# Autodesk Inventor assembly: sled
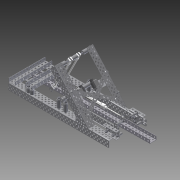
[picture p0: Inventor's stored thumbnail of the model, 180x180]
Saved by Autodesk Inventor 2014 SP1 (Build 180222100, 222)
## iProperties
Created: 2014-02-27
Part Number: sled
Document SubType Name: Assembly
Designer: Ryan
Author: Ryan
## Documents named in this file (36)
- C:\Users\Ryan\Desktop\sw\toss up 5th A bot\intake\sled.iam
- C:\Users\Ryan\Desktop\sw\lib\Aperture VEX CAD Library\Standoffs\BEAM-0500.ipt
- C:\Users\Ryan\Desktop\sw\lib\Aperture VEX CAD Library\Spacers\SPACER-0500-0125.ipt
- C:\Users\Ryan\Desktop\sw\lib\Aperture VEX CAD Library\Metal\C Channel\2 x 11.ipt
- C:\Users\Ryan\Desktop\sw\lib\Aperture VEX CAD Library\Metal\vex hinge\hinge.iam
- C:\Users\Ryan\Desktop\sw\lib\Aperture VEX CAD Library\Metal\C Channel\2 x 35.ipt
- C:\Users\Ryan\Desktop\sw\lib\Aperture VEX CAD Library\Spacers\SPACER-0500-0500.ipt
- C:\Users\Ryan\Desktop\sw\lib\Aperture VEX CAD Library\Metal\L Bar\2 x 14.ipt
- C:\Users\Ryan\Desktop\sw\lib\Aperture VEX CAD Library\Hardware\8-32\8-32_.375.ipt
- C:\Users\Ryan\Desktop\sw\lib\Aperture VEX CAD Library\Metal\Custom 1 bar\4 holes.ipt
- C:\Users\Ryan\Desktop\sw\lib\Aperture VEX CAD Library\Bearing Blocks\Bearing Block.ipt
- C:\Users\Ryan\Desktop\sw\lib\Aperture VEX CAD Library\Metal\Custom 1 bar\12.ipt
- C:\Users\Ryan\Desktop\sw\lib\Aperture VEX CAD Library\Pnuematics\Solenoid, Fwd, Reverse.iam
- C:\Users\Ryan\Desktop\sw\lib\Aperture VEX CAD Library\Shaft\5.5 inch shaft.ipt
- C:\Users\Ryan\Desktop\sw\lib\Aperture VEX CAD Library\Pnuematics\Cylinder, Bi-directional.iam
- C:\Users\Ryan\Desktop\sw\lib\Aperture VEX CAD Library\Pnuematics\End Gusset Fixed.ipt
- C:\Users\Ryan\Desktop\sw\lib\Aperture VEX CAD Library\Pnuematics\Cylinder, Bi-directional-Parts\Nut 8-32 Hex.ipt
- C:\Users\Ryan\Desktop\sw\lib\Aperture VEX CAD Library\Spacers\SPACER-0500-0250.ipt
- C:\Users\Ryan\Desktop\sw\lib\Aperture VEX CAD Library\Metal\Gussets\Lockbar.ipt
- C:\Users\Ryan\Desktop\sw\lib\Aperture VEX CAD Library\Spacers\SPACER-0500-0375.ipt
- C:\Users\Ryan\Desktop\sw\lib\Aperture VEX CAD Library\Hardware\8-32\8-32 nylock.ipt
- C:\Users\Ryan\Desktop\sw\lib\Aperture VEX CAD Library\Hardware\8-32\8-32_.500.ipt
- C:\Users\Ryan\Desktop\sw\lib\Aperture VEX CAD Library\Hardware\6-32\6-32_.250.ipt
- C:\Users\Ryan\Desktop\sw\lib\Aperture VEX CAD Library\Hardware\6-32\thinner locknut.iam
- C:\Users\Ryan\Desktop\sw\lib\Aperture VEX CAD Library\Spacers\thin\SPACER-0320-00625.ipt
- C:\Users\Ryan\Desktop\sw\lib\Aperture VEX CAD Library\Bearing Blocks\Pillow Block.ipt
- C:\Users\Ryan\Desktop\sw\lib\Aperture VEX CAD Library\Hardware\Shaft Collar.ipt
- C:\Users\Ryan\Desktop\sw\lib\Aperture VEX CAD Library\Metal\C Channel\2 x 4.ipt
- C:\Users\Ryan\Desktop\sw\lib\Aperture VEX CAD Library\Hardware\8-32\8-23_.750.ipt
- C:\Users\Ryan\Desktop\sw\lib\Aperture VEX CAD Library\Spacers\thin\SPACER-0320-0500.ipt
- C:\Users\Ryan\Desktop\sw\lib\Aperture VEX CAD Library\Spacers\thin\SPACER-0320-0250.ipt
- C:\Users\Ryan\Desktop\sw\lib\Aperture VEX CAD Library\Metal\C Channel\2 x 13 sides cut off.ipt
- C:\Users\Ryan\Desktop\sw\lib\Aperture VEX CAD Library\Metal\Custom 1 bar\1 x 3.ipt
- C:\Users\Ryan\Desktop\sw\lib\Aperture VEX CAD Library\Spacers\thin\SPACER-0320-0125.ipt
- C:\Users\Ryan\Desktop\sw\lib\Aperture VEX CAD Library\Spacers\thin\SPACER-0320-0375.ipt
- C:\Users\Ryan\Desktop\sw\lib\Aperture VEX CAD Library\Metal\L Bar\2 x 30.ipt
## Components (188 placed, 35 different names)
1. 2 x 30:1 — Mate:6, Flush:1, Flush:2, Mate:29, Mate:31, Mate:32, Mate:133, Mate:217, Mate:219, Mate:244, Mate:247, Mate:400, Mate:401, Mate:402, Mate:420, Mate:421, Mate:422, Mate:423, Mate:426, Mate:476, Flush:19, Flush:20, Mate:477, Mate:529, Mate:530, Mate:531, Mate:532
2. 2 x 11:1 — Mate:6, Flush:1, Flush:2, Mate:8, Mate:9, Flush:7, Flush:8, Mate:224, Flush:17, Flush:18
3. 2 x 30:2 — Mate:8, Mate:15, Mate:17, Mate:20, Mate:39, Mate:43, Mate:44, Mate:52, Mate:54, Mate:214, Mate:215, Mate:237, Mate:238, Mate:355, Mate:356, Mate:416, Mate:419, Flush:17, Flush:18, Flush:23, Mate:519, Flush:24, Mate:523, Mate:526, Mate:527, Mate:528, Mate:535
4. hinge:1 [sub-assembly] — Mate:9, Flush:7, Flush:8, Mate:10, Flush:9, Flush:10, Mate:94, Mate:95, Mate:96, Mate:136, Mate:137, Mate:192, Mate:220, Mate:221, Mate:222, Mate:404, Mate:408
5. 2 x 35:3 — Mate:10, Flush:9, Flush:10, Flush:12, Mate:277, Mate:279, Mate:306, Mate:307, Mate:309, Mate:312, Mate:322, Mate:323, Mate:324, Mate:327, Mate:403, Mate:409
6. SPACER-0500-0500:1 — Mate:15, Mate:17, Mate:23, Mate:24, Mate:212
7. SPACER-0500-0500:2 — Mate:20, Mate:21, Mate:22, Mate:213, Mate:258, Mate:416, Mate:417, Mate:418, Mate:419
8. SPACER-0500-0125:3 — Mate:21, Mate:22
9. SPACER-0500-0125:4 — Mate:23, Mate:24, Mate:35, Mate:36, Mate:37
10. SPACER-0500-0500:3 — Mate:29, Mate:31, Mate:216, Mate:422
11. SPACER-0500-0500:4 — Mate:32, Mate:218, Mate:420, Mate:421
12. SPACER-0500-0125:5 — Mate:261
13. SPACER-0500-0125:6 — Mate:260
14. 2 x 11:2 — Mate:35, Mate:36, Mate:37, Mate:257, Mate:259, Mate:262, Mate:263, Mate:417, Mate:418
15. 2 x 14:1 — Mate:39, Mate:40, Mate:41, Mate:42, Mate:45, Mate:56, Mate:57, Mate:58, Mate:59, Mate:60, Mate:64, Mate:65, Mate:66, Mate:67, Mate:68, Angle:1, Flush:11, Mate:151, Mate:241, Mate:242, Mate:254, Mate:289, Mate:291, Mate:299, Mate:475
16. 8-32_.375:1 — Mate:40, Mate:41, Mate:42, Mate:43, Mate:44, Mate:134, Mate:239
17. 4 holes:1 — Mate:45, Mate:46, Mate:47, Mate:49, Mate:51, Mate:53, Mate:55
18. 8-32_.375:2 — Mate:46, Mate:47, Mate:49, Mate:255, Mate:475
19. 8-32_.375:3 — Mate:51, Mate:52, Mate:53, Mate:54, Mate:55, Mate:135, Mate:236
20. Bearing Block:1 — Mate:56, Mate:57, Mate:58, Mate:59, Mate:69, Mate:70, Mate:75, Mate:92, Mate:284, Mate:285, Mate:286, Mate:287, Mate:288, Mate:290
21. 12:1 — Mate:60, Mate:61, Mate:62, Mate:63, Mate:144, Mate:145, Mate:146
22. 8-32_.375:4 — Mate:61, Mate:62, Mate:63, Mate:64, Mate:65, Mate:240
23. Solenoid, Fwd, Reverse:1 [sub-assembly] — Mate:66, Mate:67, Mate:68, Angle:1, Angle:5, Mate:298, Mate:300
24. 5.5 inch shaft:1 — Flush:11, Mate:69, Mate:70
25. Cylinder, Bi-directional:1 [sub-assembly] — Mate:75, Mate:76, Mate:77, Mate:78, Mate:87, Mate:93
26. Nut 8-32 Hex:1 — Mate:185, Mate:186
27. End Gusset Fixed:2 — Mate:76, Mate:77, Mate:78, Mate:86, Mate:325, Mate:326, Mate:327, Mate:330, Mate:332
28. Nut 8-32 Hex:2 — Mate:86, Mate:87
29. SPACER-0500-0500:5 — Mate:88, Mate:89, Mate:90
30. SPACER-0500-0500:6 — Mate:89, Mate:91, Mate:92, Mate:93, Mate:132
31. SPACER-0500-0250:1 — Mate:88, Mate:90, Mate:91
32. Lockbar:1 — Mate:94, Mate:95, Mate:96, Mate:200, Mate:201, Angle:6
33. 2 x 14:2 — Mate:97, Mate:98, Mate:99, Mate:100, Mate:101, Mate:103, Mate:109, Mate:110, Mate:111, Mate:112, Mate:113, Angle:3, Mate:115, Mate:116, Mate:133, Mate:138, Mate:142, Mate:143, Mate:150, Mate:248, Mate:251, Mate:253, Mate:294, Mate:295, Mate:297
34. 8-32_.375:5 — Mate:97, Mate:98, Mate:99, Mate:134, Mate:246
35. 4 holes:2 — Mate:100, Mate:102, Mate:104, Mate:105, Mate:106, Mate:107, Mate:108
36. 8-32_.375:6 — Mate:101, Mate:102, Mate:103, Mate:104, Mate:105, Mate:250
37. 8-32_.375:7 — Mate:106, Mate:107, Mate:108, Mate:135, Mate:245
38. Bearing Block:2 — Mate:109, Mate:110, Mate:111, Mate:112, Mate:117, Mate:124, Mate:280, Mate:281, Mate:282, Mate:283, Mate:292, Mate:293
39. 12:2 — Mate:113, Mate:139, Mate:140, Mate:141, Mate:147, Mate:148, Mate:149
40. Solenoid, Fwd, Reverse:2 [sub-assembly] — Angle:3, Mate:115, Mate:116, Mate:138, Angle:5, Mate:296, Mate:302
41. Cylinder, Bi-directional:2 [sub-assembly] — Mate:117, Mate:118, Mate:119, Mate:120, Mate:123, Mate:132, Mate:185, Mate:334
42. End Gusset Fixed:3 — Mate:118, Mate:119, Mate:120, Mate:186, Mate:304, Mate:305, Mate:315, Mate:318
43. SPACER-0500-0500:7 — Mate:125, Mate:127, Mate:128, Mate:333
44. SPACER-0500-0500:8 — Mate:123, Mate:124, Mate:125, Mate:126
45. SPACER-0500-0250:2 — Mate:126, Mate:127, Mate:128
46. Lockbar:2 — Mate:136, Mate:137, Mate:189, Mate:192, Mate:193, Mate:202, Mate:203, Angle:6
47. 8-32_.375:8 — Mate:139, Mate:140, Mate:141, Mate:142, Mate:143, Mate:249
48. 8-32_.375:9 — Mate:144, Mate:145, Mate:146, Mate:150, Mate:252
49. 8-32_.375:10 — Mate:147, Mate:148, Mate:149, Mate:151, Mate:243
50. SPACER-0500-0375:1 — Mate:333, Mate:334, Mate:335, Mate:336
51. 8-32_.375:22 — Mate:200, Mate:201, Mate:276
52. 8-32_.375:23 — Mate:202, Mate:203, Mate:278, Mate:403
53. 8-32_.375:26 — Mate:304, Mate:305, Mate:306, Mate:307, Mate:308, Mate:310, Mate:311, Mate:314
54. 8-32_.375:27 — Mate:268, Mate:320, Mate:321, Mate:322, Mate:323, Mate:325, Mate:326, Mate:331
55. 8-32_.375:28 — Mate:212, Mate:215, Mate:256
56. 8-32_.375:29 — Mate:213, Mate:214
57. 8-32_.375:30 — Mate:216, Mate:217
58. 8-32_.375:31 — Mate:218, Mate:219
59. 8-32 nylock:8 — Mate:236, Mate:237
60. 8-32 nylock:9 — Mate:238, Mate:239
61. 8-32 nylock:10 — Mate:240, Mate:241
62. 8-32 nylock:11 — Mate:242, Mate:243
63. 8-32 nylock:12 — Mate:244, Mate:245
64. 8-32 nylock:13 — Mate:246, Mate:247
65. 8-32 nylock:14 — Mate:248, Mate:249
66. 8-32 nylock:15 — Mate:250, Mate:251
67. 8-32 nylock:16 — Mate:252, Mate:253
68. 8-32 nylock:17 — Mate:254, Mate:255
69. 8-32 nylock:18 — Mate:256, Mate:257
70. 8-32 nylock:19 — Mate:258, Mate:259
71. 8-32 nylock:20 — Mate:260, Mate:263
72. 8-32 nylock:21 — Mate:261, Mate:262
73. 8-32 nylock:24 — Mate:268, Mate:332
74. 8-32 nylock:34 — Mate:276, Mate:277
75. 8-32 nylock:35 — Mate:278, Mate:279
76. 8-32 nylock:36 — Mate:280, Mate:281
77. 8-32 nylock:37 — Mate:282, Mate:283
78. 8-32 nylock:38 — Mate:284, Mate:285
79. 8-32 nylock:39 — Mate:286, Mate:287
80. 8-32_.500:1 — Mate:288, Mate:289
81. 8-32_.500:2 — Mate:290, Mate:291
82. 8-32_.500:3 — Mate:293, Mate:295
83. 8-32_.500:4 — Mate:292, Mate:294
84. 6-32_.250:1 — Mate:296, Mate:297, Mate:303
85. 6-32_.250:2 — Mate:298, Mate:299, Mate:301
86. thinner locknut:1 [sub-assembly] — Mate:300, Mate:301
87. thinner locknut:2 [sub-assembly] — Mate:302, Mate:303
88. SPACER-0320-00625:1 — Mate:308, Mate:309, Mate:310
89. SPACER-0320-00625:2 — Mate:311, Mate:312, Mate:316, Mate:317
90. 8-32 nylock:40 — Mate:314, Mate:315
91. SPACER-0320-00625:3 — Mate:316, Mate:317, Mate:318
92. SPACER-0320-00625:4 — Mate:320, Mate:321, Mate:324
93. SPACER-0320-00625:5 — Mate:331
94. SPACER-0320-00625:6 — Mate:330
95. SPACER-0500-0375:2 — Mate:335, Mate:336
96. Pillow Block:1 — Mate:358, Mate:359, Mate:360, Mate:361, Mate:362, Mate:363
97. SPACER-0500-0500:10
98. SPACER-0500-0500:12
99. SPACER-0500-0500:9
100. SPACER-0500-0500:11
101. 8-32_.375:46 — Mate:355
102. 8-32_.375:47 — Mate:356
103. 8-32 nylock:41 — Mate:358, Mate:359
104. 8-32 nylock:42 — Mate:360, Mate:361
105. SPACER-0500-0500:13 — Mate:362, Mate:363, Mate:365, Mate:366
106. SPACER-0500-0500:14 — Mate:364, Mate:365, Mate:367, Mate:368, Mate:369
107. SPACER-0500-0500:15 — Mate:364, Mate:366, Mate:367
108. Shaft Collar:1 — Mate:368, Mate:369, Mate:370, Mate:371
109. SPACER-0500-0125:7 — Mate:370, Mate:371, Mate:372, Mate:373
110. Cylinder, Bi-directional:3 [sub-assembly] — Mate:372, Mate:373, Mate:396, Mate:397, Mate:411, Mate:412, Mate:413, Mate:414
111. Pillow Block:2 — Mate:374, Mate:375, Mate:376, Mate:377, Mate:378, Mate:382, Mate:383, Mate:387, Mate:398, Mate:399
112. 8-32_.375:48 — Mate:379, Mate:401
113. 8-32_.375:49 — Mate:384, Mate:402
114. 8-32 nylock:43 — Mate:374, Mate:375
115. 8-32 nylock:44 — Mate:376, Mate:377
116. SPACER-0500-0500:16 — Mate:378, Mate:380, Mate:381, Mate:399
117. SPACER-0500-0500:17 — Mate:379, Mate:380, Mate:381, Mate:400
118. SPACER-0500-0500:18 — Mate:382, Mate:383, Mate:385, Mate:386
119. SPACER-0500-0500:19 — Mate:384, Mate:385, Mate:386
120. SPACER-0500-0500:20 — Mate:387, Mate:388, Mate:390, Mate:398
121. SPACER-0500-0500:21 — Mate:388, Mate:389, Mate:391, Mate:392, Mate:393, Mate:396
122. SPACER-0500-0500:22 — Mate:389, Mate:390, Mate:391
123. Shaft Collar:2 — Mate:392, Mate:393, Mate:394, Mate:395
124. SPACER-0500-0125:8 — Mate:394, Mate:395, Mate:397
125. 8-32 nylock:45 — Mate:404, Mate:405
126. 8-32 nylock:46 — Mate:407, Mate:408
127. 8-32 nylock:47 — Mate:406, Mate:409
128. End Gusset Fixed:4 — Mate:412, Mate:413, Mate:414, Mate:415, Mate:474, Mate:478
129. Nut 8-32 Hex:3 — Mate:411, Mate:415
130. 2 x 4:1 — Mate:423, Mate:424, Mate:428, Mate:430, Mate:435, Mate:436, Mate:437, Mate:439, Mate:440, Mate:441, Mate:444, Mate:476, Flush:19, Flush:20
131. 8-32 nylock:51 — Mate:437, Mate:438
132. SPACER-0320-0500:1 — Mate:430, Mate:433, Mate:434, Mate:435, Mate:436
133. 8-23_.750:1 — Mate:433, Mate:434, Mate:438
134. 8-32 nylock:52 — Mate:439, Mate:440, Mate:441, Mate:445
135. SPACER-0320-00625:7 — Mate:442, Mate:443, Mate:448
136. SPACER-0320-0250:1 — Mate:442, Mate:443, Mate:444, Mate:445
137. 8-23_.750:2 — Mate:449, Mate:450
138. 2 x 13 sides cut off:1 — Mate:448, Mate:449, Mate:450, Mate:451, Flush:15, Flush:16, Mate:453, Mate:455, Mate:457, Mate:463, Mate:465
139. 1 x 3:1 — Mate:451, Flush:15, Flush:16, Mate:452, Mate:454, Mate:456, Mate:459, Mate:461, Mate:466, Mate:468, Mate:469
140. SPACER-0320-0125:1 — Mate:452, Mate:453, Mate:454, Mate:460
141. SPACER-0320-0125:2 — Mate:455, Mate:456, Mate:457, Mate:458
142. 8-32_.375:52 — Mate:458, Mate:459, Mate:462
143. 8-32_.375:53 — Mate:460, Mate:461, Mate:464
144. 8-32 nylock:53 — Mate:462, Mate:463
145. 8-32 nylock:54 — Mate:464, Mate:465
146. SPACER-0320-0375:1 — Mate:466, Mate:468, Mate:469, Mate:470, Mate:471, Mate:472, Mate:525
147. 8-32 nylock:55 — Mate:470, Mate:473, Mate:474, Mate:478
148. BEAM-0500:3 — Mate:471, Mate:472, Mate:473
149. 2 x 4:2 — Mate:479, Mate:480, Mate:482, Mate:483, Mate:484, Mate:485, Mate:489, Mate:490, Mate:491, Mate:493, Flush:23, Mate:519, Flush:24
150. 8-32 nylock:57 — Mate:482, Mate:486
151. SPACER-0320-0500:2 — Mate:483, Mate:484, Mate:485, Mate:487, Mate:488
152. 8-23_.750:3 — Mate:486, Mate:487, Mate:488
153. 8-32 nylock:58 — Mate:489, Mate:490, Mate:491, Mate:492
154. SPACER-0320-0250:2 — Mate:492, Mate:493, Mate:494, Mate:520, Mate:521
155. 8-23_.750:4 — Mate:494, Mate:495, Mate:496, Mate:524
156. 2 x 13 sides cut off:2 — Mate:495, Mate:496, Flush:21, Flush:22, Mate:497, Mate:499, Mate:501, Mate:503, Mate:508, Mate:510, Mate:522, Mate:524
157. 1 x 3:2 — Flush:21, Flush:22, Mate:497, Mate:498, Mate:500, Mate:502, Mate:504, Mate:506, Mate:512, Mate:513, Mate:514
158. SPACER-0320-0125:3 — Mate:498, Mate:499, Mate:500, Mate:507
159. SPACER-0320-0125:4 — Mate:501, Mate:502, Mate:503, Mate:505
160. 8-32_.375:55 — Mate:504, Mate:505, Mate:509
161. 8-32_.375:56 — Mate:506, Mate:507, Mate:511
162. 8-32 nylock:59 — Mate:508, Mate:509
163. 8-32 nylock:60 — Mate:510, Mate:511
164. SPACER-0320-0375:2 — Mate:512, Mate:513, Mate:514, Mate:515, Mate:517, Mate:518, Mate:525
165. 8-32 nylock:61 — Mate:515, Mate:516
166. BEAM-0500:4 — Mate:516, Mate:517, Mate:518
167. SPACER-0320-00625:8 — Mate:520, Mate:521, Mate:522
168. 8-32 nylock:63 — Mate:526, Mate:527, Mate:528, Mate:534
169. 8-32 nylock:64 — Mate:529, Mate:530, Mate:531, Mate:533
170. SPACER-0320-00625:9 — Mate:532, Mate:533
171. SPACER-0320-00625:10 — Mate:534, Mate:535
172. 8-32_.375:32 — Mate:220, Mate:221, Mate:222, Mate:223
173. 8-32_.375:12 — Mate:189, Mate:193, Mate:407
174. 8-32 nylock:1 — Mate:223, Mate:224
175. 8-32_.375:40
176. 8-32_.375:41 — Mate:406
177. 8-32 nylock:6
178. 8-32_.375:42
179. 8-32_.375:43 — Mate:405
180. 8-32 nylock:7
181. 8-32_.375:50 — Mate:424, Mate:426, Mate:427, Mate:477
182. 8-32 nylock:48 — Mate:427, Mate:428
183. 8-32_.375:51
184. 8-32 nylock:49
185. 8-32_.375:54 — Mate:479, Mate:481, Mate:523
186. 8-32 nylock:56 — Mate:480, Mate:481
187. 8-32_.375:57
188. 8-32 nylock:62
## Component patterns: (3 elements, first: 8-32_.375:32 + 8-32_.375:12 + 8-32 nylock:1), (2 elements, first: 8-32_.375:50 + 8-32 nylock:48), (2 elements, first: 8-32_.375:54 + 8-32 nylock:56)
## Relationships (436: Mate 414, Flush 18, Angle 4)
- Mate:6: 2 x 30:1 ↔ 2 x 11:1
- Flush:1: 2 x 30:1 ↔ 2 x 11:1
- Flush:2: 2 x 30:1 ↔ 2 x 11:1
- Mate:8: 2 x 11:1 ↔ 2 x 30:2
- Mate:9: 2 x 11:1 ↔ hinge:1
- Flush:7: 2 x 11:1 ↔ hinge:1
- Flush:8: 2 x 11:1 ↔ hinge:1
- Mate:10: hinge:1 ↔ 2 x 35:3
- Flush:9: hinge:1 ↔ 2 x 35:3
- Flush:10: hinge:1 ↔ 2 x 35:3
- Mate:15: 2 x 30:2 ↔ SPACER-0500-0500:1
- Mate:17 (2.3114 mm): 2 x 30:2 ↔ SPACER-0500-0500:1
- Mate:20: 2 x 30:2 ↔ SPACER-0500-0500:2
- Mate:21: SPACER-0500-0500:2 ↔ SPACER-0500-0125:3
- Mate:22: SPACER-0500-0500:2 ↔ SPACER-0500-0125:3
- Mate:23: SPACER-0500-0500:1 ↔ SPACER-0500-0125:4
- Mate:24: SPACER-0500-0500:1 ↔ SPACER-0500-0125:4
- [Mate]: SPACER-0500-0500:4 ↔ SPACER-0500-0125:5
- [Mate]: SPACER-0500-0500:4 ↔ SPACER-0500-0125:5
- [Mate]: SPACER-0500-0500:3 ↔ SPACER-0500-0125:6
- [Mate]: SPACER-0500-0500:3 ↔ SPACER-0500-0125:6
- Mate:29 (2.3114 mm): 2 x 30:1 ↔ SPACER-0500-0500:3
- Mate:31: 2 x 30:1 ↔ SPACER-0500-0500:3
- Mate:32: 2 x 30:1 ↔ SPACER-0500-0500:4
- Mate:35: SPACER-0500-0125:4 ↔ 2 x 11:2
- Mate:36 (2.3114 mm): SPACER-0500-0125:4 ↔ 2 x 11:2
- Mate:37 (2.3114 mm): SPACER-0500-0125:4 ↔ 2 x 11:2
- Mate:39: 2 x 30:2 ↔ 2 x 14:1
- Mate:40 (2.3114 mm): 2 x 14:1 ↔ 8-32_.375:1
- Mate:41 (2.3114 mm): 2 x 14:1 ↔ 8-32_.375:1
- Mate:42: 2 x 14:1 ↔ 8-32_.375:1
- Mate:43 (2.3114 mm): 2 x 30:2 ↔ 8-32_.375:1
- Mate:44 (-61.1886 mm): 2 x 30:2 ↔ 8-32_.375:1
- Mate:45: 2 x 14:1 ↔ 4 holes:1
- Mate:46 (2.3114 mm): 4 holes:1 ↔ 8-32_.375:2
- Mate:47 (2.3114 mm): 4 holes:1 ↔ 8-32_.375:2
- Mate:49: 4 holes:1 ↔ 8-32_.375:2
- Mate:51 (2.3114 mm): 4 holes:1 ↔ 8-32_.375:3
- Mate:52 (65.8114 mm): 2 x 30:2 ↔ 8-32_.375:3
- Mate:53 (2.3114 mm): 4 holes:1 ↔ 8-32_.375:3
- Mate:54 (2.3114 mm): 2 x 30:2 ↔ 8-32_.375:3
- Mate:55: 4 holes:1 ↔ 8-32_.375:3
- Mate:56: 2 x 14:1 ↔ Bearing Block:1
- Mate:57 (2.3114 mm): 2 x 14:1 ↔ Bearing Block:1
- Mate:58 (2.3114 mm): 2 x 14:1 ↔ Bearing Block:1
- Mate:59 (2.3114 mm): 2 x 14:1 ↔ Bearing Block:1
- Mate:60: 2 x 14:1 ↔ 12:1
- Mate:61 (2.3114 mm): 12:1 ↔ 8-32_.375:4
- Mate:62 (2.3114 mm): 12:1 ↔ 8-32_.375:4
- Mate:63: 12:1 ↔ 8-32_.375:4
- Mate:64 (2.3114 mm): 2 x 14:1 ↔ 8-32_.375:4
- Mate:65 (2.3114 mm): 2 x 14:1 ↔ 8-32_.375:4
- Mate:66: 2 x 14:1 ↔ Solenoid, Fwd, Reverse:1
- Mate:67 (2.3114 mm): 2 x 14:1 ↔ Solenoid, Fwd, Reverse:1
- Mate:68 (2.3114 mm): 2 x 14:1 ↔ Solenoid, Fwd, Reverse:1
- Angle:1 (0 deg): 2 x 14:1 ↔ Solenoid, Fwd, Reverse:1
- Flush:11: 2 x 14:1 ↔ 5.5 inch shaft:1
- Mate:69 (-1.5875 mm): Bearing Block:1 ↔ 5.5 inch shaft:1
- Mate:70 (-1.5875 mm): Bearing Block:1 ↔ 5.5 inch shaft:1
- Mate:75: Bearing Block:1 ↔ Cylinder, Bi-directional:1
- Mate:76: Cylinder, Bi-directional:1 ↔ End Gusset Fixed:2
- Mate:77 (2.3114 mm): Cylinder, Bi-directional:1 ↔ End Gusset Fixed:2
- Mate:78 (2.3114 mm): Cylinder, Bi-directional:1 ↔ End Gusset Fixed:2
- Mate:86: End Gusset Fixed:2 ↔ Nut 8-32 Hex:2
- Mate:87: Cylinder, Bi-directional:1 ↔ Nut 8-32 Hex:2
- Mate:88: SPACER-0500-0500:5 ↔ SPACER-0500-0250:1
- Mate:89: SPACER-0500-0500:5 ↔ SPACER-0500-0500:6
- Mate:90: SPACER-0500-0500:5 ↔ SPACER-0500-0250:1
- Mate:91: SPACER-0500-0500:6 ↔ SPACER-0500-0250:1
- Mate:92: Bearing Block:1 ↔ SPACER-0500-0500:6
- Mate:93: Cylinder, Bi-directional:1 ↔ SPACER-0500-0500:6
- Mate:94: hinge:1 ↔ Lockbar:1
- Mate:95 (2.3114 mm): hinge:1 ↔ Lockbar:1
- Mate:96 (2.3114 mm): hinge:1 ↔ Lockbar:1
- Flush:12 (-12.7 mm): 2 x 35:3
- Mate:97: 2 x 14:2 ↔ 8-32_.375:5
- Mate:98 (2.3114 mm): 2 x 14:2 ↔ 8-32_.375:5
- Mate:99 (2.3114 mm): 2 x 14:2 ↔ 8-32_.375:5
- Mate:100: 2 x 14:2 ↔ 4 holes:2
- Mate:101 (2.3114 mm): 2 x 14:2 ↔ 8-32_.375:6
- Mate:102: 4 holes:2 ↔ 8-32_.375:6
- Mate:103 (2.3114 mm): 2 x 14:2 ↔ 8-32_.375:6
- Mate:104 (2.3114 mm): 4 holes:2 ↔ 8-32_.375:6
- Mate:105 (2.3114 mm): 4 holes:2 ↔ 8-32_.375:6
- Mate:106: 4 holes:2 ↔ 8-32_.375:7
- Mate:107 (2.3114 mm): 4 holes:2 ↔ 8-32_.375:7
- Mate:108 (2.3114 mm): 4 holes:2 ↔ 8-32_.375:7
- Mate:109 (2.3114 mm): 2 x 14:2 ↔ Bearing Block:2
- Mate:110 (2.3114 mm): 2 x 14:2 ↔ Bearing Block:2
- Mate:111 (2.3114 mm): 2 x 14:2 ↔ Bearing Block:2
- Mate:112: 2 x 14:2 ↔ Bearing Block:2
- Mate:113: 2 x 14:2 ↔ 12:2
- Angle:3 (0 deg): 2 x 14:2 ↔ Solenoid, Fwd, Reverse:2
- Mate:115 (2.3114 mm): 2 x 14:2 ↔ Solenoid, Fwd, Reverse:2
- Mate:116: 2 x 14:2 ↔ Solenoid, Fwd, Reverse:2
- Mate:117: Bearing Block:2 ↔ Cylinder, Bi-directional:2
- Mate:118 (2.3114 mm): Cylinder, Bi-directional:2 ↔ End Gusset Fixed:3
- Mate:119 (2.3114 mm): Cylinder, Bi-directional:2 ↔ End Gusset Fixed:3
- Mate:120: Cylinder, Bi-directional:2 ↔ End Gusset Fixed:3
- Mate:123: Cylinder, Bi-directional:2 ↔ SPACER-0500-0500:8
- Mate:124: Bearing Block:2 ↔ SPACER-0500-0500:8
- Mate:125: SPACER-0500-0500:7 ↔ SPACER-0500-0500:8
- Mate:126: SPACER-0500-0500:8 ↔ SPACER-0500-0250:2
- Mate:127: SPACER-0500-0500:7 ↔ SPACER-0500-0250:2
- Mate:128: SPACER-0500-0500:7 ↔ SPACER-0500-0250:2
- Mate:132: SPACER-0500-0500:6 ↔ Cylinder, Bi-directional:2
- Mate:133: 2 x 30:1 ↔ 2 x 14:2
- Mate:134: 8-32_.375:1 ↔ 8-32_.375:5
- Mate:135: 8-32_.375:3 ↔ 8-32_.375:7
- Mate:136 (2.3114 mm): hinge:1 ↔ Lockbar:2
- Mate:137 (2.3114 mm): hinge:1 ↔ Lockbar:2
- Mate:138 (2.3114 mm): 2 x 14:2 ↔ Solenoid, Fwd, Reverse:2
- Angle:5 (0 deg): Solenoid, Fwd, Reverse:1 ↔ Solenoid, Fwd, Reverse:2
- Mate:139 (2.3114 mm): 12:2 ↔ 8-32_.375:8
- Mate:140 (2.3114 mm): 12:2 ↔ 8-32_.375:8
- Mate:141: 12:2 ↔ 8-32_.375:8
- Mate:142 (2.3114 mm): 2 x 14:2 ↔ 8-32_.375:8
- Mate:143 (2.3114 mm): 2 x 14:2 ↔ 8-32_.375:8
- Mate:144 (2.3114 mm): 12:1 ↔ 8-32_.375:9
- Mate:145 (2.3114 mm): 12:1 ↔ 8-32_.375:9
- Mate:146: 12:1 ↔ 8-32_.375:9
- Mate:147 (2.3114 mm): 12:2 ↔ 8-32_.375:10
- Mate:148 (2.3114 mm): 12:2 ↔ 8-32_.375:10
- Mate:149: 12:2 ↔ 8-32_.375:10
- Mate:150 (2.3114 mm): 2 x 14:2 ↔ 8-32_.375:9
- Mate:151 (2.3114 mm): 2 x 14:1 ↔ 8-32_.375:10
- Mate:185: Nut 8-32 Hex:1 ↔ Cylinder, Bi-directional:2
- Mate:186: Nut 8-32 Hex:1 ↔ End Gusset Fixed:3
- Mate:189: Lockbar:2 ↔ 8-32_.375:12
- Mate:192: hinge:1 ↔ Lockbar:2
- Mate:193: Lockbar:2 ↔ 8-32_.375:12
- Mate:200: Lockbar:1 ↔ 8-32_.375:22
- Mate:201: Lockbar:1 ↔ 8-32_.375:22
- Mate:202: Lockbar:2 ↔ 8-32_.375:23
- Mate:203: Lockbar:2 ↔ 8-32_.375:23
- Mate:212: SPACER-0500-0500:1 ↔ 8-32_.375:28
- Mate:213: SPACER-0500-0500:2 ↔ 8-32_.375:29
- Mate:214: 2 x 30:2 ↔ 8-32_.375:29
- Mate:215: 2 x 30:2 ↔ 8-32_.375:28
- Mate:216: SPACER-0500-0500:3 ↔ 8-32_.375:30
- Mate:217: 2 x 30:1 ↔ 8-32_.375:30
- Mate:218: SPACER-0500-0500:4 ↔ 8-32_.375:31
- Mate:219: 2 x 30:1 ↔ 8-32_.375:31
- Mate:220 (2.3114 mm): hinge:1 ↔ 8-32_.375:32
- Mate:221 (2.3114 mm): hinge:1 ↔ 8-32_.375:32
- Mate:222: hinge:1 ↔ 8-32_.375:32
- Mate:223: 8-32_.375:32 ↔ 8-32 nylock:1
- Mate:224: 2 x 11:1 ↔ 8-32 nylock:1
- Mate:236: 8-32_.375:3 ↔ 8-32 nylock:8
- Mate:237: 2 x 30:2 ↔ 8-32 nylock:8
- Mate:238: 2 x 30:2 ↔ 8-32 nylock:9
- Mate:239: 8-32_.375:1 ↔ 8-32 nylock:9
- Mate:240: 8-32_.375:4 ↔ 8-32 nylock:10
- Mate:241: 2 x 14:1 ↔ 8-32 nylock:10
- Mate:242: 2 x 14:1 ↔ 8-32 nylock:11
- Mate:243: 8-32_.375:10 ↔ 8-32 nylock:11
- Mate:244: 2 x 30:1 ↔ 8-32 nylock:12
- Mate:245: 8-32_.375:7 ↔ 8-32 nylock:12
- Mate:246: 8-32_.375:5 ↔ 8-32 nylock:13
- Mate:247: 2 x 30:1 ↔ 8-32 nylock:13
- Mate:248: 2 x 14:2 ↔ 8-32 nylock:14
- Mate:249: 8-32_.375:8 ↔ 8-32 nylock:14
- Mate:250: 8-32_.375:6 ↔ 8-32 nylock:15
- Mate:251: 2 x 14:2 ↔ 8-32 nylock:15
- Mate:252: 8-32_.375:9 ↔ 8-32 nylock:16
- Mate:253: 2 x 14:2 ↔ 8-32 nylock:16
- Mate:254: 2 x 14:1 ↔ 8-32 nylock:17
- Mate:255: 8-32_.375:2 ↔ 8-32 nylock:17
- Mate:256: 8-32_.375:28 ↔ 8-32 nylock:18
- Mate:257: 2 x 11:2 ↔ 8-32 nylock:18
- Mate:258: SPACER-0500-0500:2 ↔ 8-32 nylock:19
- Mate:259: 2 x 11:2 ↔ 8-32 nylock:19
- Mate:260: SPACER-0500-0125:6 ↔ 8-32 nylock:20
- Mate:261: SPACER-0500-0125:5 ↔ 8-32 nylock:21
- Mate:262: 2 x 11:2 ↔ 8-32 nylock:21
- Mate:263: 2 x 11:2 ↔ 8-32 nylock:20
- Mate:268: 8-32_.375:27 ↔ 8-32 nylock:24
- Mate:276: 8-32_.375:22 ↔ 8-32 nylock:34
- Mate:277: 2 x 35:3 ↔ 8-32 nylock:34
- Mate:278: 8-32_.375:23 ↔ 8-32 nylock:35
- Mate:279: 2 x 35:3 ↔ 8-32 nylock:35
- Mate:280: Bearing Block:2 ↔ 8-32 nylock:36
- Mate:281: Bearing Block:2 ↔ 8-32 nylock:36
- Mate:282: Bearing Block:2 ↔ 8-32 nylock:37
- Mate:283: Bearing Block:2 ↔ 8-32 nylock:37
- Mate:284: Bearing Block:1 ↔ 8-32 nylock:38
- Mate:285: Bearing Block:1 ↔ 8-32 nylock:38
- Mate:286: Bearing Block:1 ↔ 8-32 nylock:39
- Mate:287: Bearing Block:1 ↔ 8-32 nylock:39
- Mate:288: Bearing Block:1 ↔ 8-32_.500:1
- Mate:289: 2 x 14:1 ↔ 8-32_.500:1
- Mate:290: Bearing Block:1 ↔ 8-32_.500:2
- Mate:291: 2 x 14:1 ↔ 8-32_.500:2
- Mate:292: Bearing Block:2 ↔ 8-32_.500:4
- Mate:293: Bearing Block:2 ↔ 8-32_.500:3
- Mate:294: 2 x 14:2 ↔ 8-32_.500:4
- Mate:295: 2 x 14:2 ↔ 8-32_.500:3
- Mate:296: Solenoid, Fwd, Reverse:2 ↔ 6-32_.250:1
- Mate:297: 2 x 14:2 ↔ 6-32_.250:1
- Mate:298: Solenoid, Fwd, Reverse:1 ↔ 6-32_.250:2
- Mate:299: 2 x 14:1 ↔ 6-32_.250:2
- Mate:300: Solenoid, Fwd, Reverse:1 ↔ thinner locknut:1
- Mate:301: 6-32_.250:2 ↔ thinner locknut:1
- Mate:302: Solenoid, Fwd, Reverse:2 ↔ thinner locknut:2
- Mate:303: 6-32_.250:1 ↔ thinner locknut:2
- Mate:304 (2.3114 mm): End Gusset Fixed:3 ↔ 8-32_.375:26
- Mate:305 (2.3114 mm): End Gusset Fixed:3 ↔ 8-32_.375:26
- Mate:306 (2.3114 mm): 2 x 35:3 ↔ 8-32_.375:26
- Mate:307 (2.3114 mm): 2 x 35:3 ↔ 8-32_.375:26
- Mate:308: 8-32_.375:26 ↔ SPACER-0320-00625:1
- Mate:309: 2 x 35:3 ↔ SPACER-0320-00625:1
- Mate:310: 8-32_.375:26 ↔ SPACER-0320-00625:1
- Mate:311: 8-32_.375:26 ↔ SPACER-0320-00625:2
- Mate:312: 2 x 35:3 ↔ SPACER-0320-00625:2
- Mate:314: 8-32_.375:26 ↔ 8-32 nylock:40
- Mate:315: End Gusset Fixed:3 ↔ 8-32 nylock:40
- Mate:316: SPACER-0320-00625:2 ↔ SPACER-0320-00625:3
- Mate:317: SPACER-0320-00625:2 ↔ SPACER-0320-00625:3
- Mate:318: End Gusset Fixed:3 ↔ SPACER-0320-00625:3
- Mate:320: 8-32_.375:27 ↔ SPACER-0320-00625:4
- Mate:321: 8-32_.375:27 ↔ SPACER-0320-00625:4
- Mate:322 (2.3114 mm): 2 x 35:3 ↔ 8-32_.375:27
- Mate:323 (2.3114 mm): 2 x 35:3 ↔ 8-32_.375:27
- Mate:324: 2 x 35:3 ↔ SPACER-0320-00625:4
- Mate:325 (2.3114 mm): End Gusset Fixed:2 ↔ 8-32_.375:27
- Mate:326 (2.3114 mm): End Gusset Fixed:2 ↔ 8-32_.375:27
- Mate:327 (3.175 mm): 2 x 35:3 ↔ End Gusset Fixed:2
- [Mate]: SPACER-0320-00625:5 ↔ SPACER-0320-00625:6
- [Mate]: SPACER-0320-00625:5 ↔ SPACER-0320-00625:6
- Mate:330: End Gusset Fixed:2 ↔ SPACER-0320-00625:6
- Mate:331: 8-32_.375:27 ↔ SPACER-0320-00625:5
- Mate:332: End Gusset Fixed:2 ↔ 8-32 nylock:24
- Mate:333: SPACER-0500-0500:7 ↔ SPACER-0500-0375:1
- Mate:334 (0.2286 mm): Cylinder, Bi-directional:2 ↔ SPACER-0500-0375:1
- Mate:335: SPACER-0500-0375:1 ↔ SPACER-0500-0375:2
- Mate:336: SPACER-0500-0375:1 ↔ SPACER-0500-0375:2
- [Mate]: 2 x 30:2 ↔ SPACER-0500-0500:10
- [Mate] (2.3114 mm): 2 x 30:2 ↔ SPACER-0500-0500:10
- [Mate] (-61.1886 mm): 2 x 30:2 ↔ SPACER-0500-0500:10
- [Mate] (2.3114 mm): 2 x 30:2 ↔ SPACER-0500-0500:12
- [Mate]: 2 x 30:2 ↔ SPACER-0500-0500:12
- [Mate] (-61.1886 mm): 2 x 30:2 ↔ SPACER-0500-0500:12
- [Mate]: SPACER-0500-0500:10 ↔ SPACER-0500-0500:9
- [Mate]: SPACER-0500-0500:10 ↔ SPACER-0500-0500:9
- [Mate]: SPACER-0500-0500:12 ↔ SPACER-0500-0500:11
- [Mate]: SPACER-0500-0500:12 ↔ SPACER-0500-0500:11
- [Mate]: Pillow Block:1 ↔ SPACER-0500-0500:11
- [Mate]: Pillow Block:1 ↔ SPACER-0500-0500:11
- [Mate]: Pillow Block:1 ↔ SPACER-0500-0500:9
- [Mate]: SPACER-0500-0500:10 ↔ 8-32_.375:46
- Mate:355: 2 x 30:2 ↔ 8-32_.375:46
- Mate:356: 2 x 30:2 ↔ 8-32_.375:47
- [Mate]: SPACER-0500-0500:12 ↔ 8-32_.375:47
- Mate:358: Pillow Block:1 ↔ 8-32 nylock:41
- Mate:359: Pillow Block:1 ↔ 8-32 nylock:41
- Mate:360: Pillow Block:1 ↔ 8-32 nylock:42
- Mate:361: Pillow Block:1 ↔ 8-32 nylock:42
- Mate:362: Pillow Block:1 ↔ SPACER-0500-0500:13
- Mate:363: Pillow Block:1 ↔ SPACER-0500-0500:13
- Mate:364: SPACER-0500-0500:14 ↔ SPACER-0500-0500:15
- Mate:365: SPACER-0500-0500:13 ↔ SPACER-0500-0500:14
- Mate:366: SPACER-0500-0500:13 ↔ SPACER-0500-0500:15
- Mate:367: SPACER-0500-0500:14 ↔ SPACER-0500-0500:15
- Mate:368: SPACER-0500-0500:14 ↔ Shaft Collar:1
- Mate:369: SPACER-0500-0500:14 ↔ Shaft Collar:1
- Mate:370: Shaft Collar:1 ↔ SPACER-0500-0125:7
- Mate:371: Shaft Collar:1 ↔ SPACER-0500-0125:7
- Mate:372: SPACER-0500-0125:7 ↔ Cylinder, Bi-directional:3
- Mate:373: SPACER-0500-0125:7 ↔ Cylinder, Bi-directional:3
- Mate:374: Pillow Block:2 ↔ 8-32 nylock:43
- Mate:375: Pillow Block:2 ↔ 8-32 nylock:43
- Mate:376: Pillow Block:2 ↔ 8-32 nylock:44
- Mate:377: Pillow Block:2 ↔ 8-32 nylock:44
- Mate:378: Pillow Block:2 ↔ SPACER-0500-0500:16
- Mate:379: 8-32_.375:48 ↔ SPACER-0500-0500:17
- Mate:380: SPACER-0500-0500:16 ↔ SPACER-0500-0500:17
- Mate:381: SPACER-0500-0500:16 ↔ SPACER-0500-0500:17
- Mate:382: Pillow Block:2 ↔ SPACER-0500-0500:18
- Mate:383: Pillow Block:2 ↔ SPACER-0500-0500:18
- Mate:384: 8-32_.375:49 ↔ SPACER-0500-0500:19
- Mate:385: SPACER-0500-0500:18 ↔ SPACER-0500-0500:19
- Mate:386: SPACER-0500-0500:18 ↔ SPACER-0500-0500:19
- Mate:387: Pillow Block:2 ↔ SPACER-0500-0500:20
- Mate:388: SPACER-0500-0500:20 ↔ SPACER-0500-0500:21
- Mate:389: SPACER-0500-0500:21 ↔ SPACER-0500-0500:22
- Mate:390: SPACER-0500-0500:20 ↔ SPACER-0500-0500:22
- Mate:391: SPACER-0500-0500:21 ↔ SPACER-0500-0500:22
- Mate:392: SPACER-0500-0500:21 ↔ Shaft Collar:2
- Mate:393: SPACER-0500-0500:21 ↔ Shaft Collar:2
- Mate:394: Shaft Collar:2 ↔ SPACER-0500-0125:8
- Mate:395: Shaft Collar:2 ↔ SPACER-0500-0125:8
- Mate:396: Cylinder, Bi-directional:3 ↔ SPACER-0500-0500:21
- Mate:397: Cylinder, Bi-directional:3 ↔ SPACER-0500-0125:8
- Mate:398: Pillow Block:2 ↔ SPACER-0500-0500:20
- Mate:399: Pillow Block:2 ↔ SPACER-0500-0500:16
- Mate:400: 2 x 30:1 ↔ SPACER-0500-0500:17
- Mate:401: 2 x 30:1 ↔ 8-32_.375:48
- Mate:402: 2 x 30:1 ↔ 8-32_.375:49
- Mate:403 (16.1036 mm): 2 x 35:3 ↔ 8-32_.375:23
- Mate:404: hinge:1 ↔ 8-32 nylock:45
- Mate:405: 8-32 nylock:45 ↔ 8-32_.375:43
- Mate:406: 8-32 nylock:47 ↔ 8-32_.375:41
- Mate:407: 8-32 nylock:46 ↔ 8-32_.375:12
- Mate:408: hinge:1 ↔ 8-32 nylock:46
- Mate:409: 2 x 35:3 ↔ 8-32 nylock:47
- Angle:6 (0 deg): Lockbar:1 ↔ Lockbar:2
- Mate:411: Cylinder, Bi-directional:3 ↔ Nut 8-32 Hex:3
- Mate:412: Cylinder, Bi-directional:3 ↔ End Gusset Fixed:4
- Mate:413 (2.3114 mm): Cylinder, Bi-directional:3 ↔ End Gusset Fixed:4
- Mate:414 (2.3114 mm): Cylinder, Bi-directional:3 ↔ End Gusset Fixed:4
- Mate:415: End Gusset Fixed:4 ↔ Nut 8-32 Hex:3
- Mate:416 (2.3114 mm): 2 x 30:2 ↔ SPACER-0500-0500:2
- Mate:417 (2.3114 mm): SPACER-0500-0500:2 ↔ 2 x 11:2
- Mate:418 (2.3114 mm): SPACER-0500-0500:2 ↔ 2 x 11:2
- Mate:419 (65.8114 mm): 2 x 30:2 ↔ SPACER-0500-0500:2
- Mate:420 (2.3114 mm): 2 x 30:1 ↔ SPACER-0500-0500:4
- Mate:421 (2.3114 mm): 2 x 30:1 ↔ SPACER-0500-0500:4
- Mate:422 (2.3114 mm): 2 x 30:1 ↔ SPACER-0500-0500:3
- Mate:423: 2 x 30:1 ↔ 2 x 4:1
- Mate:424 (2.3114 mm): 2 x 4:1 ↔ 8-32_.375:50
- Mate:426: 2 x 30:1 ↔ 8-32_.375:50
- Mate:427: 8-32_.375:50 ↔ 8-32 nylock:48
- Mate:428: 2 x 4:1 ↔ 8-32 nylock:48
- Mate:430: 2 x 4:1 ↔ SPACER-0320-0500:1
- Mate:433: SPACER-0320-0500:1 ↔ 8-23_.750:1
- Mate:434: SPACER-0320-0500:1 ↔ 8-23_.750:1
- Mate:435 (2.3114 mm): 2 x 4:1 ↔ SPACER-0320-0500:1
- Mate:436 (2.3114 mm): 2 x 4:1 ↔ SPACER-0320-0500:1
- Mate:437: 2 x 4:1 ↔ 8-32 nylock:51
- Mate:438: 8-32 nylock:51 ↔ 8-23_.750:1
- Mate:439 (2.3114 mm): 2 x 4:1 ↔ 8-32 nylock:52
- Mate:440 (2.3114 mm): 2 x 4:1 ↔ 8-32 nylock:52
- Mate:441: 2 x 4:1 ↔ 8-32 nylock:52
- Mate:442: SPACER-0320-00625:7 ↔ SPACER-0320-0250:1
- Mate:443: SPACER-0320-00625:7 ↔ SPACER-0320-0250:1
- Mate:444: 2 x 4:1 ↔ SPACER-0320-0250:1
- Mate:445: 8-32 nylock:52 ↔ SPACER-0320-0250:1
- [Mate]: SPACER-0320-0250:1 ↔ 8-23_.750:2
- [Mate] (1.1684 mm): SPACER-0320-00625:7 ↔ 8-23_.750:2
- Mate:448: SPACER-0320-00625:7 ↔ 2 x 13 sides cut off:1
- Mate:449 (2.3114 mm): 8-23_.750:2 ↔ 2 x 13 sides cut off:1
- Mate:450 (2.3114 mm): 8-23_.750:2 ↔ 2 x 13 sides cut off:1
- Mate:451: 2 x 13 sides cut off:1 ↔ 1 x 3:1
- Flush:15: 2 x 13 sides cut off:1 ↔ 1 x 3:1
- Flush:16: 2 x 13 sides cut off:1 ↔ 1 x 3:1
- Mate:452 (2.3114 mm): 1 x 3:1 ↔ SPACER-0320-0125:1
- Mate:453: 2 x 13 sides cut off:1 ↔ SPACER-0320-0125:1
- Mate:454 (2.3114 mm): 1 x 3:1 ↔ SPACER-0320-0125:1
- Mate:455 (2.3114 mm): 2 x 13 sides cut off:1 ↔ SPACER-0320-0125:2
- Mate:456 (2.3114 mm): 1 x 3:1 ↔ SPACER-0320-0125:2
- Mate:457: 2 x 13 sides cut off:1 ↔ SPACER-0320-0125:2
- Mate:458: SPACER-0320-0125:2 ↔ 8-32_.375:52
- Mate:459: 1 x 3:1 ↔ 8-32_.375:52
- Mate:460: SPACER-0320-0125:1 ↔ 8-32_.375:53
- Mate:461: 1 x 3:1 ↔ 8-32_.375:53
- Mate:462: 8-32_.375:52 ↔ 8-32 nylock:53
- Mate:463: 2 x 13 sides cut off:1 ↔ 8-32 nylock:53
- Mate:464: 8-32_.375:53 ↔ 8-32 nylock:54
- Mate:465: 2 x 13 sides cut off:1 ↔ 8-32 nylock:54
- Mate:466 (2.3114 mm): 1 x 3:1 ↔ SPACER-0320-0375:1
- Mate:468 (2.3114 mm): 1 x 3:1 ↔ SPACER-0320-0375:1
- Mate:469: 1 x 3:1 ↔ SPACER-0320-0375:1
- Mate:470: SPACER-0320-0375:1 ↔ 8-32 nylock:55
- Mate:471: SPACER-0320-0375:1 ↔ BEAM-0500:3
- Mate:472: SPACER-0320-0375:1 ↔ BEAM-0500:3
- Mate:473: 8-32 nylock:55 ↔ BEAM-0500:3
- Mate:474 (2.3114 mm): End Gusset Fixed:4 ↔ 8-32 nylock:55
- Flush:17: 2 x 11:1 ↔ 2 x 30:2
- Flush:18: 2 x 11:1 ↔ 2 x 30:2
- Mate:475 (2.3114 mm): 2 x 14:1 ↔ 8-32_.375:2
- Mate:476: 2 x 30:1 ↔ 2 x 4:1
- Flush:19: 2 x 30:1 ↔ 2 x 4:1
- Flush:20: 2 x 30:1 ↔ 2 x 4:1
- Mate:477 (2.3114 mm): 2 x 30:1 ↔ 8-32_.375:50
- Mate:478 (2.3114 mm): End Gusset Fixed:4 ↔ 8-32 nylock:55
- Mate:479 (2.3114 mm): 2 x 4:2 ↔ 8-32_.375:54
- Mate:480: 2 x 4:2 ↔ 8-32 nylock:56
- Mate:481: 8-32_.375:54 ↔ 8-32 nylock:56
- Mate:482: 2 x 4:2 ↔ 8-32 nylock:57
- Mate:483 (2.3114 mm): 2 x 4:2 ↔ SPACER-0320-0500:2
- Mate:484 (2.3114 mm): 2 x 4:2 ↔ SPACER-0320-0500:2
- Mate:485: 2 x 4:2 ↔ SPACER-0320-0500:2
- Mate:486: 8-32 nylock:57 ↔ 8-23_.750:3
- Mate:487: SPACER-0320-0500:2 ↔ 8-23_.750:3
- Mate:488: SPACER-0320-0500:2 ↔ 8-23_.750:3
- Mate:489: 2 x 4:2 ↔ 8-32 nylock:58
- Mate:490 (2.3114 mm): 2 x 4:2 ↔ 8-32 nylock:58
- Mate:491 (2.3114 mm): 2 x 4:2 ↔ 8-32 nylock:58
- Mate:492: 8-32 nylock:58 ↔ SPACER-0320-0250:2
- Mate:493: 2 x 4:2 ↔ SPACER-0320-0250:2
- Mate:494: SPACER-0320-0250:2 ↔ 8-23_.750:4
- Mate:495 (2.3114 mm): 8-23_.750:4 ↔ 2 x 13 sides cut off:2
- Mate:496 (2.3114 mm): 8-23_.750:4 ↔ 2 x 13 sides cut off:2
- Flush:21: 2 x 13 sides cut off:2 ↔ 1 x 3:2
- Flush:22: 2 x 13 sides cut off:2 ↔ 1 x 3:2
- Mate:497: 2 x 13 sides cut off:2 ↔ 1 x 3:2
- Mate:498 (2.3114 mm): 1 x 3:2 ↔ SPACER-0320-0125:3
- Mate:499: 2 x 13 sides cut off:2 ↔ SPACER-0320-0125:3
- Mate:500 (2.3114 mm): 1 x 3:2 ↔ SPACER-0320-0125:3
- Mate:501: 2 x 13 sides cut off:2 ↔ SPACER-0320-0125:4
- Mate:502 (2.3114 mm): 1 x 3:2 ↔ SPACER-0320-0125:4
- Mate:503 (2.3114 mm): 2 x 13 sides cut off:2 ↔ SPACER-0320-0125:4
- Mate:504: 1 x 3:2 ↔ 8-32_.375:55
- Mate:505: SPACER-0320-0125:4 ↔ 8-32_.375:55
- Mate:506: 1 x 3:2 ↔ 8-32_.375:56
- Mate:507: SPACER-0320-0125:3 ↔ 8-32_.375:56
- Mate:508: 2 x 13 sides cut off:2 ↔ 8-32 nylock:59
- Mate:509: 8-32_.375:55 ↔ 8-32 nylock:59
- Mate:510: 2 x 13 sides cut off:2 ↔ 8-32 nylock:60
- Mate:511: 8-32_.375:56 ↔ 8-32 nylock:60
- Mate:512: 1 x 3:2 ↔ SPACER-0320-0375:2
- Mate:513 (2.3114 mm): 1 x 3:2 ↔ SPACER-0320-0375:2
- Mate:514 (2.3114 mm): 1 x 3:2 ↔ SPACER-0320-0375:2
- Mate:515: SPACER-0320-0375:2 ↔ 8-32 nylock:61
- Mate:516: 8-32 nylock:61 ↔ BEAM-0500:4
- Mate:517: SPACER-0320-0375:2 ↔ BEAM-0500:4
- Mate:518: SPACER-0320-0375:2 ↔ BEAM-0500:4
- Flush:23: 2 x 30:2 ↔ 2 x 4:2
- Mate:519: 2 x 30:2 ↔ 2 x 4:2
- Flush:24: 2 x 30:2 ↔ 2 x 4:2
- Mate:520: SPACER-0320-0250:2 ↔ SPACER-0320-00625:8
- Mate:521: SPACER-0320-0250:2 ↔ SPACER-0320-00625:8
- Mate:522: 2 x 13 sides cut off:2 ↔ SPACER-0320-00625:8
- Mate:523: 2 x 30:2 ↔ 8-32_.375:54
- Mate:524: 8-23_.750:4 ↔ 2 x 13 sides cut off:2
- Mate:525: SPACER-0320-0375:1 ↔ SPACER-0320-0375:2
- Mate:526: 2 x 30:2 ↔ 8-32 nylock:63
- Mate:527 (2.3114 mm): 2 x 30:2 ↔ 8-32 nylock:63
- Mate:528 (2.3114 mm): 2 x 30:2 ↔ 8-32 nylock:63
- Mate:529: 2 x 30:1 ↔ 8-32 nylock:64
- Mate:530 (2.3114 mm): 2 x 30:1 ↔ 8-32 nylock:64
- Mate:531 (2.3114 mm): 2 x 30:1 ↔ 8-32 nylock:64
- Mate:532: 2 x 30:1 ↔ SPACER-0320-00625:9
- Mate:533: 8-32 nylock:64 ↔ SPACER-0320-00625:9
- Mate:534: 8-32 nylock:63 ↔ SPACER-0320-00625:10
- Mate:535: 2 x 30:2 ↔ SPACER-0320-00625:10
## Named parameters: q = 2.3114 mm, d34_d30 = 0 mm, d35_d31 = 0 mm, d36_d32 = 0 mm, d37_d33 = 0 mm, d381_d367 = 0 mm, d382_d368 = 0 mm
